# Autodesk Inventor assembly: R-wing
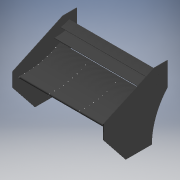
[picture p0: Inventor's stored thumbnail of the model, 180x180]
Saved by Autodesk Inventor 2018.1 (Build 221171000, 171)
## iProperties
Created: 2017-10-22
Part Number: R-wing
Material: 一般
Document SubType Name: Assembly
Designer: ku_sk
Mass: 8773.72 g
Surface Area: 41617.1 cm^2
Volume: 5548.68 cm^3
Density: 1.58123 g/cm^3
Author: ku_sk
## Documents named in this file (8)
- D:\kuwano\Documents\Inventor\KITformula\KS-15_Aero_CAD\type4\R-wing\R-wing.iam
- D:\kuwano\Documents\Inventor\KITformula\KS-15_Aero_CAD\type4\R-wing\parts\element_base.ipt
- D:\kuwano\Documents\Inventor\KITformula\KS-15_Aero_CAD\type4\R-wing\parts\carbon_pipe_φ20.ipt
- D:\kuwano\Documents\Inventor\KITformula\KS-15_Aero_CAD\type4\R-wing\parts\end_plate.ipt
- D:\kuwano\Documents\Inventor\KITformula\KS-15_Aero_CAD\type4\R-wing\parts\element_r_1.ipt
- D:\kuwano\Documents\Inventor\KITformula\KS-15_Aero_CAD\type4\R-wing\parts\element_r_2.ipt
- D:\kuwano\Documents\Inventor\KITformula\KS-15_Aero_CAD\type4\R-wing\parts\element_clip.ipt
- D:\kuwano\Documents\Inventor\KITformula\KS-15_Aero_CAD\type4\R-wing\parts\cover.ipt
## Components (20 placed, 7 different names)
1. element_base:1 — メイト:2, メイト:6, メイト:7, メイト:8, メイト:10, メイト:47
2. element_base:2 — メイト:3, メイト:6, メイト:8, メイト:9, メイト:14, メイト:15, メイト:48
3. element_base:3 — メイト:1, メイト:2, メイト:3, メイト:4, メイト:5, メイト:9, メイト:17
4. element_base:4 — メイト:1, メイト:4, メイト:5, メイト:7, メイト:10, メイト:11, メイト:12, メイト:13, フラッシュ:1, フラッシュ:2, フラッシュ:3, メイト:16, フラッシュ:6
5. carbon_pipe_φ20:1 — メイト:11, フラッシュ:1, メイト:18
6. carbon_pipe_φ20:2 — メイト:12, フラッシュ:2, メイト:14
7. carbon_pipe_φ20:3 — メイト:13, フラッシュ:3, メイト:15
8. end_plate:1 — メイト:17, フラッシュ:4, フラッシュ:5, メイト:29, メイト:30, メイト:39, メイト:40
9. end_plate:2 — メイト:16, フラッシュ:4, フラッシュ:5, メイト:19, メイト:20, メイト:23, メイト:24, メイト:37, メイト:38, メイト:45, メイト:46
10. element_r_1:1 — メイト:19, メイト:21, メイト:22, メイト:25, メイト:26, メイト:27, メイト:28, メイト:31, メイト:32
11. element_r_2:1 — メイト:20, メイト:33, メイト:34, メイト:35, メイト:36, メイト:41, メイト:42, メイト:43, メイト:44
12. cover:1 — メイト:47, メイト:48, フラッシュ:6
13. element_clip:1 — メイト:28, メイト:29, メイト:31
14. element_clip:2 — メイト:27, メイト:30, メイト:32
15. element_clip:3 — メイト:22, メイト:23, メイト:26
16. element_clip:4 — メイト:21, メイト:24, メイト:25, メイト:46
17. element_clip:5 — メイト:33, メイト:38, メイト:44, メイト:45
18. element_clip:6 — メイト:34, メイト:37, メイト:43
19. element_clip:7 — メイト:36, メイト:40, メイト:41
20. element_clip:8 — メイト:35, メイト:39, メイト:42
## Relationships (54: Mate 48, Flush 6)
- メイト:1 [Mate]: element_base:3 ↔ element_base:4
- メイト:2 [Mate]: element_base:1 ↔ element_base:3
- メイト:3 [Mate]: element_base:2 ↔ element_base:3
- メイト:4 [Mate] (960 mm): element_base:3 ↔ element_base:4
- メイト:5 [Mate]: element_base:3 ↔ element_base:4
- メイト:6 [Mate] (316.6667 mm): element_base:1 ↔ element_base:2
- メイト:7 [Mate] (316.667 mm): element_base:1 ↔ element_base:4
- メイト:8 [Mate]: element_base:1 ↔ element_base:2
- メイト:9 [Mate]: element_base:2 ↔ element_base:3
- メイト:10 [Mate]: element_base:1 ↔ element_base:4
- メイト:11 [Mate]: element_base:4 ↔ carbon_pipe_φ20:1
- メイト:12 [Mate]: element_base:4 ↔ carbon_pipe_φ20:2
- メイト:13 [Mate]: element_base:4 ↔ carbon_pipe_φ20:3
- フラッシュ:1 [Flush]: element_base:4 ↔ carbon_pipe_φ20:1
- フラッシュ:2 [Flush]: element_base:4 ↔ carbon_pipe_φ20:2
- フラッシュ:3 [Flush]: element_base:4 ↔ carbon_pipe_φ20:3
- メイト:14 [Mate]: element_base:2 ↔ carbon_pipe_φ20:2
- メイト:15 [Mate]: element_base:2 ↔ carbon_pipe_φ20:3
- メイト:16 [Mate]: element_base:4 ↔ end_plate:2
- メイト:17 [Mate]: element_base:3 ↔ end_plate:1
- フラッシュ:4 [Flush]: end_plate:1 ↔ end_plate:2
- フラッシュ:5 [Flush]: end_plate:1 ↔ end_plate:2
- メイト:18 [Mate]: carbon_pipe_φ20:1
- メイト:19 [Mate]: end_plate:2 ↔ element_r_1:1
- メイト:20 [Mate]: end_plate:2 ↔ element_r_2:1
- メイト:21 [Mate]: element_r_1:1 ↔ element_clip:4
- メイト:22 [Mate]: element_r_1:1 ↔ element_clip:3
- メイト:23 [Mate]: end_plate:2 ↔ element_clip:3
- メイト:24 [Mate]: end_plate:2 ↔ element_clip:4
- メイト:25 [Mate]: element_r_1:1 ↔ element_clip:4
- メイト:26 [Mate]: element_r_1:1 ↔ element_clip:3
- メイト:27 [Mate]: element_r_1:1 ↔ element_clip:2
- メイト:28 [Mate]: element_r_1:1 ↔ element_clip:1
- メイト:29 [Mate]: end_plate:1 ↔ element_clip:1
- メイト:30 [Mate]: end_plate:1 ↔ element_clip:2
- メイト:31 [Mate]: element_r_1:1 ↔ element_clip:1
- メイト:32 [Mate]: element_r_1:1 ↔ element_clip:2
- メイト:33 [Mate]: element_r_2:1 ↔ element_clip:5
- メイト:34 [Mate]: element_r_2:1 ↔ element_clip:6
- メイト:35 [Mate]: element_r_2:1 ↔ element_clip:8
- メイト:36 [Mate]: element_r_2:1 ↔ element_clip:7
- メイト:37 [Mate]: end_plate:2 ↔ element_clip:6
- メイト:38 [Mate]: end_plate:2 ↔ element_clip:5
- メイト:39 [Mate]: end_plate:1 ↔ element_clip:8
- メイト:40 [Mate]: end_plate:1 ↔ element_clip:7
- メイト:41 [Mate]: element_r_2:1 ↔ element_clip:7
- メイト:42 [Mate]: element_r_2:1 ↔ element_clip:8
- メイト:43 [Mate]: element_r_2:1 ↔ element_clip:6
- メイト:44 [Mate]: element_r_2:1 ↔ element_clip:5
- メイト:45 [Mate]: end_plate:2 ↔ element_clip:5
- メイト:46 [Mate]: end_plate:2 ↔ element_clip:4
- メイト:47 [Mate]: element_base:1 ↔ cover:1
- メイト:48 [Mate]: element_base:2 ↔ cover:1
- フラッシュ:6 [Flush]: element_base:4 ↔ cover:1
